# Autodesk Inventor assembly: 3.157 roller
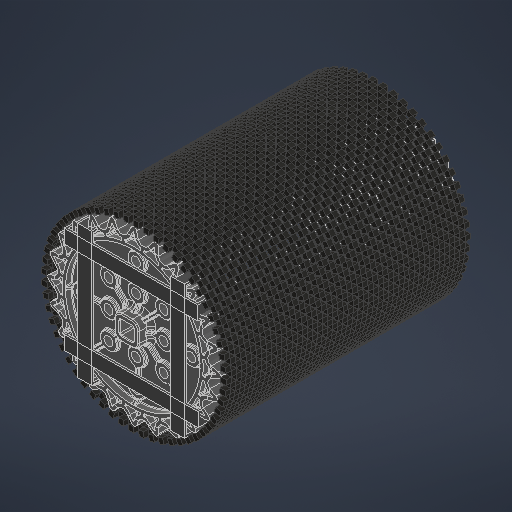
[picture p0: Inventor's stored thumbnail of the model, 512x512]
Saved by Autodesk Inventor 2025.2 (Build 292293000, 293)
## iProperties
Created: 2025-12-04
Part Number: 3.157 roller
Document SubType Name: Assembly
Designer: cloudy
Mass: 88.161 g
Surface Area: 1448.02 cm^2
Volume: 75.6051 cm^3
Density: 1.16607 g/cm^3
Author: cloudy
## Documents named in this file (5)
- C:\Users\cloudy\Documents\GitHub\aura-cad\15\3.157 roller.iam
- C:\Users\cloudy\Documents\GitHub\aura-cad\!lib\Motion\Sprockets\9P Sprocket.iam
- C:\Users\cloudy\Documents\GitHub\aura-cad\!lib\Motion\Sprockets\9P Sprocket\9P 24T Sprocket, No Insert.iam
- C:\Users\cloudy\Documents\GitHub\aura-cad\15\mesh 3.157.ipt
- C:\Users\cloudy\Documents\GitHub\aura-cad\15\band.ipt
## Components (7 placed, 3 different names)
1. 9P 24T Sprocket, No Insert:1 [sub-assembly] — Insert:1, Mate:1, Insert:3, Mate:2
2. 9P 24T Sprocket, No Insert:2 [sub-assembly] — Insert:1, Mate:1
3. mesh 3.157:1 — Insert:3
4. band:1 — Flush:3
5. band:2 — Flush:1
6. band:3 — Mate:2, Flush:1, Flush:2
7. band:4 — Flush:2, Flush:3
## Relationships (7: Flush 3, Insert 2, Mate 2)
- Insert:1 (101.6 mm): 9P 24T Sprocket, No Insert:1 ↔ 9P 24T Sprocket, No Insert:2
- Mate:1: 9P 24T Sprocket, No Insert:1 ↔ 9P 24T Sprocket, No Insert:2
- Insert:3 (-0.508 mm): 9P 24T Sprocket, No Insert:1 ↔ mesh 3.157:1
- Mate:2: 9P 24T Sprocket, No Insert:1 ↔ band:3
- Flush:1: band:2 ↔ band:3
- Flush:2: band:3 ↔ band:4
- Flush:3: band:1 ↔ band:4
